# Autodesk Inventor assembly: ConveyorBaseAssembly
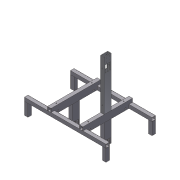
[picture p0: Inventor's stored thumbnail of the model, 180x180]
Saved by Autodesk Inventor 2012 (Build 160160000, 160)
## iProperties
Created: 2012-01-21
Part Number: ConveyorBaseAssembly
Document SubType Name: Assembly
Designer: JesseK
Author: JesseK
## Documents named in this file (4)
- Z:\UserData\Documents\Inventor\team1885frc\Robot2012\ConveyorBase\ConveyorBaseAssembly.iam
- Z:\UserData\Documents\Inventor\team1885frc\Robot2012\Drawings\ConveyorDriveSide_20Jan.iam
- Z:\UserData\Documents\Inventor\team1885frc\Robot2012\Drawings\ConveyorIdleSide_20Jan.iam
- Z:\UserData\Documents\Inventor\team1885frc\Robot2012\Drawings\ConveyorCrossFrame_20Jan.iam
## Components (4 placed, 3 different names)
1. ConveyorDriveSide_20Jan:1 [sub-assembly] — Mate:2, Flush:1, Mate:4, Mate:5, Mate:6, Mate:7
2. ConveyorIdleSide_20Jan:1 [sub-assembly] — Mate:1, Mate:3, Mate:4
3. ConveyorCrossFrame_20Jan:1 [sub-assembly] — Mate:1, Mate:2, Mate:3, Flush:1, Mate:5, Flush:2
4. ConveyorCrossFrame_20Jan:2 [sub-assembly] — Mate:6, Flush:2, Mate:7
## Relationships (9: Mate 7, Flush 2)
- Mate:1: ConveyorIdleSide_20Jan:1 ↔ ConveyorCrossFrame_20Jan:1
- Mate:2: ConveyorDriveSide_20Jan:1 ↔ ConveyorCrossFrame_20Jan:1
- Mate:3: ConveyorIdleSide_20Jan:1 ↔ ConveyorCrossFrame_20Jan:1
- Flush:1: ConveyorDriveSide_20Jan:1 ↔ ConveyorCrossFrame_20Jan:1
- Mate:4 (203.2 mm): ConveyorDriveSide_20Jan:1 ↔ ConveyorIdleSide_20Jan:1
- Mate:5 (-165.1 mm): ConveyorDriveSide_20Jan:1 ↔ ConveyorCrossFrame_20Jan:1
- Mate:6: ConveyorDriveSide_20Jan:1 ↔ ConveyorCrossFrame_20Jan:2
- Flush:2: ConveyorCrossFrame_20Jan:1 ↔ ConveyorCrossFrame_20Jan:2
- Mate:7: ConveyorDriveSide_20Jan:1 ↔ ConveyorCrossFrame_20Jan:2
